# Autodesk Inventor assembly: pince
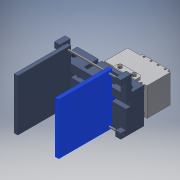
[picture p0: Inventor's stored thumbnail of the model, 180x180]
Saved by Autodesk Inventor 2017 (Build 210142000, 142)
## iProperties
Part Number: pince
Material: Générique
Document SubType Name: Assembly
Designer: Biscuit
Author: Biscuit
## Documents named in this file (6)
- C:\Users\Biscuit\Google Drive\ENSEIRB\EIRBOT\COUPE 2018\Cubes\pince.iam
- C:\Users\Biscuit\Google Drive\ENSEIRB\EIRBOT\COUPE 2018\Cubes\SupportPlateau.ipt
- C:\Users\Biscuit\Google Drive\ENSEIRB\EIRBOT\COUPE 2018\Cubes\extremite_pince.ipt
- C:\Users\Biscuit\Google Drive\ENSEIRB\EIRBOT\COUPE 2018\Cubes\ax12.iam
- C:\Users\Biscuit\Google Drive\ENSEIRB\EIRBOT\COUPE 2018\Cubes\pince\Design Accelerator\Arbre3.iam
- C:\Users\Biscuit\Google Drive\ENSEIRB\EIRBOT\COUPE 2018\Cubes\pince\Design Accelerator\Arbre5.iam
## Components (6 placed, 4 different names)
1. SupportPlateau:1 — Placage:1, Placage:2, Placage:3, Placage:4, Placage:5, Angle:1, Placage:10, Placage:11, Angle:2
2. extremite_pince:1 — Placage:8, Placage:12
3. extremite_pince:2 — Placage:9, Placage:13
4. ax12:1 [sub-assembly] — Placage:1, Placage:2, Placage:3
5. Arbre:1 [sub-assembly] — Placage:4, Placage:5, Angle:1, Placage:8, Placage:9
6. Arbre:2 [sub-assembly] — Placage:10, Placage:11, Angle:2, Placage:12, Placage:13
## Relationships (13: Mate 11, Angle 2)
- Placage:1 [Mate]: SupportPlateau:1 ↔ ax12:1
- Placage:2 [Mate]: SupportPlateau:1 ↔ ax12:1
- Placage:3 [Mate]: SupportPlateau:1 ↔ ax12:1
- Placage:4 [Mate]: SupportPlateau:1 ↔ Arbre:1
- Placage:5 [Mate]: SupportPlateau:1 ↔ Arbre:1
- Angle:1 (0 deg): SupportPlateau:1 ↔ Arbre:1
- Placage:8 [Mate]: extremite_pince:1 ↔ Arbre:1
- Placage:9 [Mate]: extremite_pince:2 ↔ Arbre:1
- Placage:10 [Mate]: SupportPlateau:1 ↔ Arbre:2
- Placage:11 [Mate]: SupportPlateau:1 ↔ Arbre:2
- Angle:2 (0 deg): SupportPlateau:1 ↔ Arbre:2
- Placage:12 [Mate]: extremite_pince:1 ↔ Arbre:2
- Placage:13 [Mate]: extremite_pince:2 ↔ Arbre:2
